# Autodesk Inventor assembly: Slab Mount Assembly - Fabricated - V1
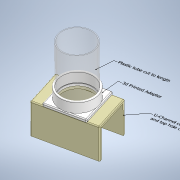
[picture p0: Inventor's stored thumbnail of the model, 180x180]
Saved by Autodesk Inventor 2022 (Build 260153000, 153)
## iProperties
Created: 2021-10-28
Part Number: Slab Mount Assembly - Fabricated - V1
Document SubType Name: Assembly
Designer: Caleb
Author: Caleb
## Documents named in this file (4)
- C:\Users\Caleb\Desktop\nebraska-silicon-lab\Hardware\MilliQan\PMT Mounts\Slab Mount - Fabricated - V1\Slab Mount Assembly - Fabricated - V1.iam
- C:\Users\Caleb\Desktop\nebraska-silicon-lab\Hardware\MilliQan\PMT Mounts\Slab Mount - Fabricated - V1\U Channel.ipt
- C:\Users\Caleb\Desktop\nebraska-silicon-lab\Hardware\MilliQan\PMT Mounts\Slab Mount - Fabricated - V1\8585K291_Impact-Resistant Polycarbonate Round Tube.ipt
- C:\Users\Caleb\Desktop\nebraska-silicon-lab\Hardware\MilliQan\PMT Mounts\Slab Mount - Fabricated - V1\Adapter.ipt
## Components (3 placed, 3 different names)
1. U Channel:1 — Angle:1, Insert:1
2. 8585K291_Impact-Resistant Polycarbonate Round Tube:1 — Insert:2
3. Adapter:1 — Angle:1, Insert:1, Insert:2
## Relationships (3: Insert 2, Angle 1)
- Angle:1 (0 deg): U Channel:1 ↔ Adapter:1
- Insert:1: U Channel:1 ↔ Adapter:1
- Insert:2: 8585K291_Impact-Resistant Polycarbonate Round Tube:1 ↔ Adapter:1
